# Autodesk Inventor assembly: 1Servo_Module_HXT
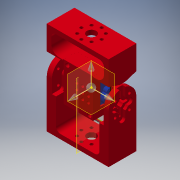
[picture p0: Inventor's stored thumbnail of the model, 180x180]
Saved by Autodesk Inventor 2019 (Build 230136000, 136)
## iProperties
Created: 2016-10-24
Part Number: 1Servo_Module_HXT
Document SubType Name: Assembly
Designer: Lucas
Author: Lucas
## Documents named in this file (11)
- D:\PhD\EDMO\EDMO_GIT\EDMO_V1-0\EDMOV1-0 Inventor\EDMO_Module_TGY_50090M.iam
- D:\PhD\Teaching\RES and Projects Construction\CAD_Files\EDMO_Module_TGY_50090M\Workspace\DIN 125 - A 3,2.ipt
- D:\PhD\Teaching\RES and Projects Construction\CAD_Files\EDMO_Module_TGY_50090M\Workspace\DIN 985 - M3.ipt
- D:\PhD\Teaching\RES and Projects Construction\CAD_Files\EDMO_Module_TGY_50090M\Workspace\DIN 912 - M2 x 0,4 x 20 x 19.ipt
- D:\PhD\Teaching\RES and Projects Construction\CAD_Files\EDMO_Module_TGY_50090M\Workspace\DIN 912 - M3 x 0,5 x 20 x 18,75.ipt
- D:\PhD\Teaching\RES and Projects Construction\CAD_Files\EDMO_Module_TGY_50090M\Workspace\Turnigy TGY-50090M Analog Servo.ipt
- D:\PhD\Teaching\RES and Projects Construction\CAD_Files\EDMO_Module_TGY_50090M\Workspace\Servo_Horn_Cross_TGY.ipt
- D:\PhD\Teaching\RES and Projects Construction\CAD_Files\EDMO_Module_TGY_50090M\Workspace\spirol_pn_151048.ipt
- D:\PhD\Teaching\RES and Projects Construction\CAD_Files\EDMO_Module_TGY_50090M\Workspace\EDMO1-0_Body.ipt
- D:\PhD\Teaching\RES and Projects Construction\CAD_Files\EDMO_Module_TGY_50090M\Workspace\EDMO1-0_Cover.ipt
- D:\PhD\Teaching\RES and Projects Construction\CAD_Files\EDMO_Module_TGY_50090M\Workspace\EDMO1-0_Arm.ipt
## Components (17 placed, 10 different names)
1. EDMO1-0_Body:1 — Insert:4, Insert:5, Mate:5, Mate:6, Flush:4, Insert:110, Insert:111, Angle:2, Insert:112, Angle:3, Flush:5, Mate:8
2. EDMO1-0_Arm:1 — Angle:4, Insert:114, Insert:115, Flush:5
3. EDMO1-0_Cover:1 — Insert:59, Insert:60, Flush:4, Angle:2, Insert:112, Angle:3
4. Turnigy TGY-50090M Analog Servo:1 — Mate:5, Mate:6, Mate:7, Flush:3, Mate:8
5. Servo_Horn_Cross_TGY:1 — Mate:7, Flush:3, Angle:4
6. spirol_pn_151048:2 — Insert:111
7. spirol_pn_151048:3 — Insert:110
8. DIN 125-1 A A 3,2:1 — Insert:4, Insert:106
9. DIN 125-1 A A 3,2:2 — Insert:5, Insert:7
10. DIN 985 - replaced by DIN EN ISO 10511 M3:1 — Insert:7, Insert:10
11. DIN 985 - replaced by DIN EN ISO 10511 M3:2 — Insert:10, Insert:48
12. DIN 125-1 A A 3,2:3 — Insert:48, Insert:115
13. DIN 125-1 A A 3,2:20 — Insert:34, Insert:114
14. DIN 985 - replaced by DIN EN ISO 10511 M3:3 — Insert:34
15. DIN 912 - replaced by DIN EN ISO 4762 M2 x 20:2 — Insert:59
16. DIN 912 - replaced by DIN EN ISO 4762 M2 x 20:3 — Insert:60
17. DIN 912 - replaced by DIN EN ISO 4762 M3 x 20:1 — Insert:106
## Relationships (24: Insert 14, Mate 4, Flush 3, Angle 3)
- Insert:4: EDMO1-0_Body:1 ↔ DIN 125-1 A A 3,2:1
- Insert:5: EDMO1-0_Body:1 ↔ DIN 125-1 A A 3,2:2
- Insert:7: DIN 125-1 A A 3,2:2 ↔ DIN 985 - replaced by DIN EN ISO 10511 M3:1
- Insert:10: DIN 985 - replaced by DIN EN ISO 10511 M3:1 ↔ DIN 985 - replaced by DIN EN ISO 10511 M3:2
- Insert:34: DIN 125-1 A A 3,2:20 ↔ DIN 985 - replaced by DIN EN ISO 10511 M3:3
- Insert:48: DIN 985 - replaced by DIN EN ISO 10511 M3:2 ↔ DIN 125-1 A A 3,2:3
- Insert:59: EDMO1-0_Cover:1 ↔ DIN 912 - replaced by DIN EN ISO 4762 M2 x 20:2
- Insert:60: EDMO1-0_Cover:1 ↔ DIN 912 - replaced by DIN EN ISO 4762 M2 x 20:3
- Insert:106: DIN 125-1 A A 3,2:1 ↔ DIN 912 - replaced by DIN EN ISO 4762 M3 x 20:1
- Mate:5: EDMO1-0_Body:1 ↔ Turnigy TGY-50090M Analog Servo:1
- Mate:6: EDMO1-0_Body:1 ↔ Turnigy TGY-50090M Analog Servo:1
- Mate:7: Turnigy TGY-50090M Analog Servo:1 ↔ Servo_Horn_Cross_TGY:1
- Flush:3 (-5 mm): Turnigy TGY-50090M Analog Servo:1 ↔ Servo_Horn_Cross_TGY:1
- Flush:4: EDMO1-0_Body:1 ↔ EDMO1-0_Cover:1
- Insert:110: EDMO1-0_Body:1 ↔ spirol_pn_151048:3
- Insert:111: EDMO1-0_Body:1 ↔ spirol_pn_151048:2
- Angle:2 (0 deg): EDMO1-0_Body:1 ↔ EDMO1-0_Cover:1
- Insert:112: EDMO1-0_Body:1 ↔ EDMO1-0_Cover:1
- Angle:3 (0 deg): EDMO1-0_Body:1 ↔ EDMO1-0_Cover:1
- Angle:4 (90 deg): EDMO1-0_Arm:1 ↔ Servo_Horn_Cross_TGY:1
- Insert:114: EDMO1-0_Arm:1 ↔ DIN 125-1 A A 3,2:20
- Insert:115: EDMO1-0_Arm:1 ↔ DIN 125-1 A A 3,2:3
- Flush:5: EDMO1-0_Body:1 ↔ EDMO1-0_Arm:1
- Mate:8 (0.2 mm): EDMO1-0_Body:1 ↔ Turnigy TGY-50090M Analog Servo:1
